# Autodesk Inventor assembly: placa_galbena_composita
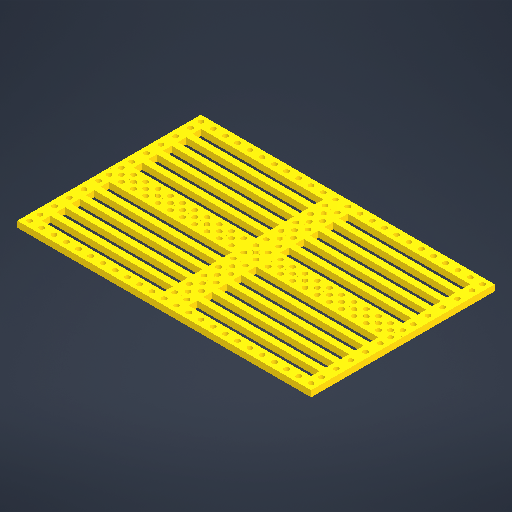
[picture p0: Inventor's stored thumbnail of the model, 512x512]
Saved by Autodesk Inventor 2026.1 (Build 301233000, 233)
## iProperties
Created: 2025-09-17
Part Number: placa_galbena_composita
Document SubType Name: Assembly
Designer: emanuel
Author: emanuel
## Documents named in this file (2)
- C:\Users\emanuel\UnFolder\SpiderRobo\3dmodel\yellow_base.iam
- C:\Users\emanuel\UnFolder\SpiderRobo\3dmodel\yellow_base_part.ipt
## Components (4 placed, 1 different names)
1. yellow_base_part:1 — Mate:2, Flush:3, Flush:4, Mate:3, Flush:5, Flush:6
2. yellow_base_part:2 — Mate:1, Flush:1, Flush:2
3. yellow_base_part:3 — Mate:1, Flush:1, Flush:2, Mate:3, Flush:5, Flush:6
4. yellow_base_part:4 — Mate:2, Flush:3, Flush:4
## Relationships (9: Flush 6, Mate 3)
- Mate:1: yellow_base_part:2 ↔ yellow_base_part:3
- Flush:1: yellow_base_part:2 ↔ yellow_base_part:3
- Flush:2: yellow_base_part:2 ↔ yellow_base_part:3
- Mate:2: yellow_base_part:1 ↔ yellow_base_part:4
- Flush:3: yellow_base_part:1 ↔ yellow_base_part:4
- Flush:4: yellow_base_part:1 ↔ yellow_base_part:4
- Mate:3: yellow_base_part:1 ↔ yellow_base_part:3
- Flush:5: yellow_base_part:1 ↔ yellow_base_part:3
- Flush:6: yellow_base_part:1 ↔ yellow_base_part:3
